# Autodesk Inventor assembly: subsystem 3 assembly
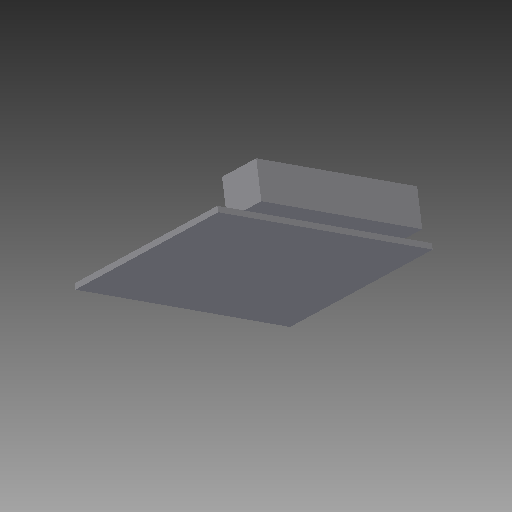
[picture p0: Inventor's stored thumbnail of the model, 512x512]
Saved by Autodesk Inventor 2019 (Build 230136000, 136)
## iProperties
Created: 2020-02-19
Part Number: subsystem 3 assembly
Document SubType Name: Assembly
Designer: User
Author: User
## Documents named in this file (3)
- C:\Users\User\Desktop\Subsystem 3\subsystem 3 assembly.iam
- C:\Users\User\Desktop\Subsystem 3\EE_Container.ipt
- C:\Users\User\Desktop\Subsystem 3\Base.ipt
## Components (2 placed, 2 different names)
1. EE_Container:1 — Rigid:1, Mate:1
2. Base:1 — Rigid:1, Mate:1
## Relationships (2: WeldJoint 1, Mate 1)
- Rigid:1 [WeldJoint]: EE_Container:1 ↔ Base:1
- Mate:1: EE_Container:1 ↔ Base:1
